# Autodesk Inventor assembly: wildfire
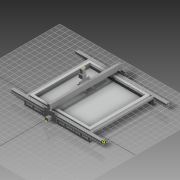
[picture p0: Inventor's stored thumbnail of the model, 180x180]
Saved by Autodesk Inventor 2013 (Build 170138000, 138)
## iProperties
Created: 2012-11-30
Part Number: wildfire
Document SubType Name: Assembly
Designer: istvan.burbank
Mass: 35060.2 g
Surface Area: 149069 cm^2
Volume: 21794.8 cm^3
Density: 1.60865 g/cm^3
Author: istvan.burbank
## Documents named in this file (6)
- D:\GitHub\Crown-Fire\CAD\wildfire.iam
- D:\GitHub\Crown-Fire\CAD\Frame\frame.iam
- D:\GitHub\Crown-Fire\CAD\GantryMount\tractor.iam
- D:\GitHub\Crown-Fire\CAD\Gantry\gantry.iam
- D:\GitHub\Crown-Fire\CAD\Carriage\carriage.iam
- D:\GitHub\Crown-Fire\CAD\CuttingHead\CuttingHead.iam
## Components (6 placed, 5 different names)
1. frame:1 [sub-assembly] — Tangent:1, Tangent:2, Tangent:3, Tangent:4, Tangent:5, Tangent:6
2. tractor:1 [sub-assembly] — Tangent:1, Tangent:2, Tangent:3, Mate:1, Mate:2
3. tractor:2 [sub-assembly] — Tangent:4, Tangent:5, Tangent:6, Mate:3, Mate:4
4. gantry:1 [sub-assembly] — Mate:1, Mate:2, Mate:3, Mate:4, Tangent:7, Tangent:8, Tangent:9
5. carriage:1 [sub-assembly] — Tangent:7, Tangent:8, Tangent:9, Mate:5
6. CuttingHead:1 [sub-assembly] — Mate:5
## Relationships (14: Tangent 9, Mate 5)
- Tangent:1: frame:1 ↔ tractor:1
- Tangent:2: frame:1 ↔ tractor:1
- Tangent:3: frame:1 ↔ tractor:1
- Tangent:4: frame:1 ↔ tractor:2
- Tangent:5: frame:1 ↔ tractor:2
- Tangent:6: frame:1 ↔ tractor:2
- Mate:1: tractor:1 ↔ gantry:1
- Mate:2: tractor:1 ↔ gantry:1
- Mate:3: tractor:2 ↔ gantry:1
- Mate:4: tractor:2 ↔ gantry:1
- Tangent:7: gantry:1 ↔ carriage:1
- Tangent:8: gantry:1 ↔ carriage:1
- Tangent:9: gantry:1 ↔ carriage:1
- Mate:5: carriage:1 ↔ CuttingHead:1
